# Autodesk Inventor assembly: Rack_assembly
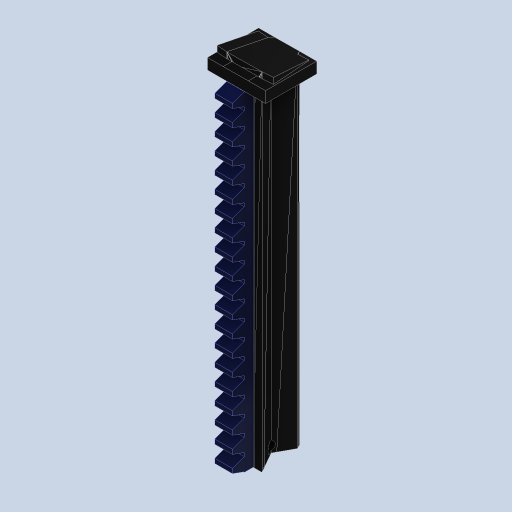
[picture p0: Inventor's stored thumbnail of the model, 512x512]
Saved by Autodesk Inventor 2023.1 (Build 271208000, 208)
## iProperties
Created: 2024-08-02
Part Number: Rack_assembly
Document SubType Name: Assembly
Designer: huchonms
Engineer: vikt
Mass: 78.3974 g
Surface Area: 71.5808 cm^2
Volume: 9.98693 cm^3
Density: 7.85 g/cm^3
tc_part_rev_length: 16.45
tc_part_rev_width: 17.93
tc_part_rev_height: 98
tc_part_rev_uom_length: mm
tc_part_rev_volume: 9987
tc_part_rev_uom_volume: mm^3
tc_part_rev_mass: 0.08
tc_part_rev_uom_mass: kg
NOV_FileName: Rack_assembly
Author: huchonms
Revision Number: 0
## Documents named in this file (3)
- C:\VaultWork\Designs\_Scratch_\Marius Huchon\Sommerprosjekt_filer\Heis deler\Actuator_Servo\Inventor\Rack_assembly.iam
- C:\VaultWork\Designs\_Scratch_\Marius Huchon\Sommerprosjekt_filer\Heis deler\Actuator_Servo\Inventor\Gammel rack.ipt
- C:\VaultWork\Designs\_Scratch_\Marius Huchon\Sommerprosjekt_filer\Heis deler\Actuator_Servo\Inventor\Rack_Dimensnjonert.ipt
## Components (2 placed, 2 different names)
1. Gammel rack:1 — Mate:1, Mate:2
2. Rack_Dimensnjonert:1 — Mate:1, Mate:2
## Relationships (2: Mate 2)
- Mate:1: Gammel rack:1 ↔ Rack_Dimensnjonert:1
- Mate:2: Gammel rack:1 ↔ Rack_Dimensnjonert:1
